# Autodesk Inventor assembly: tirette
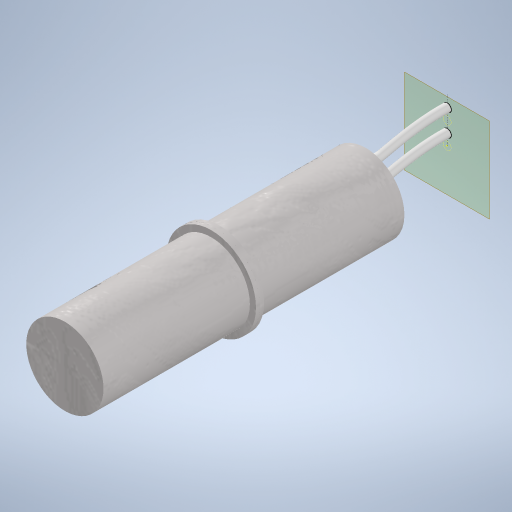
[picture p0: Inventor's stored thumbnail of the model, 512x512]
Saved by Autodesk Inventor 2024.2 (Build 282272000, 272)
## iProperties
Created: 2023-11-11
Part Number: tirette
Document SubType Name: Assembly
Designer: adrie
Author: adrie
## Documents named in this file (3)
- C:\Users\adrie\Desktop\meca_robotbebou\tirette\tirette.iam
- C:\Users\adrie\Desktop\meca_robotbebou\tirette\capteur_tirette_fixe.ipt
- C:\Users\adrie\Desktop\meca_robotbebou\tirette\capteur_tirette_mobile.ipt
## Components (2 placed, 2 different names)
1. capteur_tirette_fixe:1 — Mate:1, Mate:2
2. capteur_tirette_mobile:1 — Mate:1, Mate:2
## Relationships (2: Mate 2)
- Mate:1: capteur_tirette_fixe:1 ↔ capteur_tirette_mobile:1
- Mate:2: capteur_tirette_fixe:1 ↔ capteur_tirette_mobile:1
